# Autodesk Inventor assembly: 122
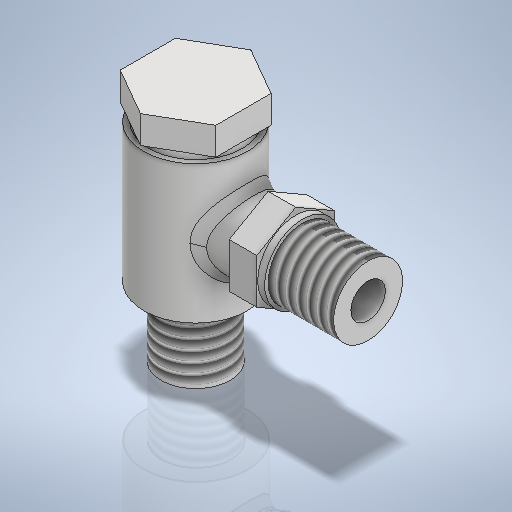
[picture p0: Inventor's stored thumbnail of the model, 512x512]
Saved by Autodesk Inventor 2025.1 (Build 291241000, 241)
## iProperties
Created: 2024-08-22
Part Number: 122
Document SubType Name: Assembly
Designer: ffogue
Author: ffogue
## Documents named in this file (3)
- C:\Projkete - Übungen\Freedom\122.iam
- C:\Projkete - Übungen\Freedom\123.ipt
- C:\Projkete - Übungen\Freedom\122 cap.ipt
## Components (2 placed, 2 different names)
1. 123:1 — Mate:1, Insert:1
2. 122 cap:1 — Mate:1, Insert:1
## Relationships (2: Mate 1, Insert 1)
- Mate:1: 123:1 ↔ 122 cap:1
- Insert:1: 123:1 ↔ 122 cap:1
